# Autodesk Inventor assembly: Custom_Delta_Assembly
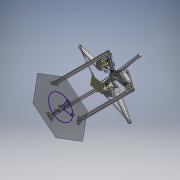
[picture p0: Inventor's stored thumbnail of the model, 180x180]
Saved by Autodesk Inventor 2019.4 (Build 234330000, 330)
## iProperties
Created: 2019-07-06
Part Number: Custom_Delta_Assembly
Document SubType Name: Assembly
Designer: Jorian Brusind
Author: Jorian Brusind
## Documents named in this file (16)
- C:\Users\Jorian Bruslind\Documents\GitHub\ECE44x_Senior_Design\Design files\Delta Robot Arm\Inventor Files\Custom_Delta\Custom_Delta_Assembly.iam
- C:\Users\Jorian Bruslind\Documents\GitHub\ECE44x_Senior_Design\Design files\Delta Robot Arm\Inventor Files\Custom_Delta\Stepper_Face.ipt
- C:\Users\Jorian Bruslind\Documents\GitHub\ECE44x_Senior_Design\Design files\Delta Robot Arm\Inventor Files\Custom_Delta\Delta_Arm.ipt
- C:\Users\Jorian Bruslind\Documents\GitHub\ECE44x_Senior_Design\Design files\Delta Robot Arm\Inventor Files\Custom_Delta\Delta_Top.ipt
- C:\Users\Jorian Bruslind\Documents\GitHub\ECE44x_Senior_Design\Design files\Delta Robot Arm\Inventor Files\McMaster Files\59935K140_METRIC BALL JOINT ROD END.ipt
- C:\Users\Jorian Bruslind\Documents\GitHub\ECE44x_Senior_Design\Design files\PetriFilm\PetriFilm.iam
- C:\Users\Jorian Bruslind\Documents\GitHub\ECE44x_Senior_Design\Design files\Delta Robot Arm\Inventor Files\McMaster Files\5537T501_ALUMINUM T-SLOTTED FRAMING EXTRUSION.ipt
- C:\Users\Jorian Bruslind\Documents\GitHub\ECE44x_Senior_Design\Design files\Delta Robot Arm\Inventor Files\McMaster Files\5537T518_T-SLOTTED FRAMING.ipt
- C:\Users\Jorian Bruslind\Documents\GitHub\ECE44x_Senior_Design\Design files\Delta Robot Arm\Inventor Files\McMaster Files\6In_ALUMINUM T-SLOTTED FRAMING EXTRUSION.ipt
- C:\Users\Jorian Bruslind\Documents\GitHub\ECE44x_Senior_Design\Design files\Delta Robot Arm\Inventor Files\McMaster Files\98861A050_LOW-STRENGTH STEEL THREADED ROD.ipt
- C:\Users\Jorian Bruslind\Documents\GitHub\ECE44x_Senior_Design\Design files\Delta Robot Arm\Inventor Files\Custom_Delta\Custom_Delta_End_Effector.ipt
- C:\Users\Jorian Bruslind\Documents\GitHub\ECE44x_Senior_Design\Design files\Delta Robot Arm\Inventor Files\Custom_Delta\80_20_Connector.ipt
- C:\Users\Jorian Bruslind\Documents\GitHub\ECE44x_Senior_Design\Design files\Delta Robot Arm\Inventor Files\Custom_Delta\NEMA17_Stepper_CL42H60.ipt
- C:\Users\Jorian Bruslind\Documents\GitHub\ECE44x_Senior_Design\Design files\Delta Robot Arm\Inventor Files\Stepper_Collar\products\12196\step\model.ipt
- C:\Users\Jorian Bruslind\Documents\GitHub\ECE44x_Senior_Design\Design files\Delta Robot Arm\Inventor Files\raspberry-pi-camera-module-v2-1.snapshot.3\RspCameraMia.iam
- C:\Users\Jorian Bruslind\Documents\GitHub\ECE44x_Senior_Design\Design files\Delta Robot Arm\Inventor Files\Custom_Delta\80_20_Connector_Bot.ipt
## Components (51 placed, 15 different names)
1. Stepper_Face:1 — Mate:126, Flush:20, Flush:23, Mate:210, Mate:211, Mate:212, Mate:216
2. Delta_Arm:1 — Mate:145, Mate:146, Mate:147, Mate:148, Mate:214, Mate:215, Mate:254
3. Stepper_Face:2 — Mate:125, Flush:18, Flush:24, Mate:222, Mate:227, Mate:230, Mate:231
4. Delta_Arm:2 — Mate:149, Mate:150, Mate:151, Mate:152, Mate:220, Mate:221, Mate:253
5. Stepper_Face:3 — Mate:127, Flush:21, Flush:22, Mate:217, Mate:218, Mate:226, Mate:228
6. Delta_Arm:3 — Mate:137, Mate:138, Mate:139, Mate:140, Mate:224, Mate:225, Mate:229
7. Delta_Top:1 — Mate:103, Mate:105, Mate:106, Mate:107, Mate:109, Mate:110, Mate:111, Mate:112, Mate:113, Mate:182, Mate:189, Mate:190, Mate:191, Mate:192, Mate:238, Mate:240, Mate:241, Mate:243, Mate:244, Mate:246
8. 59935K140_METRIC BALL JOINT ROD END:2 — Mate:145, Mate:146, Mate:159, Mate:160
9. 59935K140_METRIC BALL JOINT ROD END:3 — Mate:151, Mate:152, Mate:153, Mate:154
10. 59935K140_METRIC BALL JOINT ROD END:5 — Mate:137, Mate:138, Mate:143, Mate:144
11. 59935K140_METRIC BALL JOINT ROD END:6 — Mate:139, Mate:140, Mate:141, Mate:142
12. 59935K140_METRIC BALL JOINT ROD END:7 — Mate:147, Mate:148, Mate:157, Mate:158
13. 59935K140_METRIC BALL JOINT ROD END:8 — Mate:149, Mate:150, Mate:155, Mate:156
14. PetriFilm:1 [sub-assembly] — Mate:181, Mate:183
15. 5537T518_T-SLOTTED FRAMING:1 — Mate:106, Mate:107, Mate:119
16. 5537T518_T-SLOTTED FRAMING:2 — Mate:103, Mate:105, Mate:118
17. 5537T518_T-SLOTTED FRAMING:3 — Mate:109, Mate:110, Mate:117
18. 6In_ALUMINUM T-SLOTTED FRAMING EXTRUSION:1 — Flush:5, Mate:121, Flush:6, Mate:126, Flush:20, Flush:23, Mate:188, Mate:235, Mate:247
19. 6In_ALUMINUM T-SLOTTED FRAMING EXTRUSION:2 — Flush:9, Flush:10, Mate:123, Mate:125, Flush:18, Flush:24, Mate:237
20. 6In_ALUMINUM T-SLOTTED FRAMING EXTRUSION:3 — Flush:7, Flush:8, Mate:122, Mate:127, Flush:21, Flush:22, Mate:233
21. 5537T501_ALUMINUM T-SLOTTED FRAMING EXTRUSION:1 — Mate:112, Mate:118, Flush:5, Mate:121, Flush:6, Mate:192, Mate:234, Flush:26, Mate:245
22. 5537T501_ALUMINUM T-SLOTTED FRAMING EXTRUSION:2 — Mate:111, Mate:119, Flush:7, Flush:8, Mate:122, Mate:190, Mate:232, Flush:25, Mate:239
23. 5537T501_ALUMINUM T-SLOTTED FRAMING EXTRUSION:3 — Mate:113, Mate:117, Flush:9, Flush:10, Mate:123, Mate:191, Mate:236, Flush:27, Mate:242
24. 98861A050_LOW-STRENGTH STEEL THREADED ROD:1 — Mate:143, Mate:144, Mate:163, Mate:164
25. 98861A050_LOW-STRENGTH STEEL THREADED ROD:2 — Mate:153, Mate:154, Mate:168, Mate:170
26. 98861A050_LOW-STRENGTH STEEL THREADED ROD:3 — Mate:155, Mate:156, Mate:167, Mate:169
27. 98861A050_LOW-STRENGTH STEEL THREADED ROD:4 — Mate:141, Mate:142, Mate:161, Mate:162
28. 98861A050_LOW-STRENGTH STEEL THREADED ROD:5 — Mate:157, Mate:158, Mate:165, Mate:172
29. 98861A050_LOW-STRENGTH STEEL THREADED ROD:6 — Mate:159, Mate:160, Mate:166, Mate:171
30. 59935K140_METRIC BALL JOINT ROD END:9 — Mate:165, Mate:172, Mate:174, Mate:178
31. 59935K140_METRIC BALL JOINT ROD END:10 — Mate:163, Mate:164, Mate:176
32. 59935K140_METRIC BALL JOINT ROD END:11 — Mate:166, Mate:171, Mate:174
33. 59935K140_METRIC BALL JOINT ROD END:12 — Mate:161, Mate:162, Mate:176, Mate:180
34. 59935K140_METRIC BALL JOINT ROD END:13 — Mate:168, Mate:170, Mate:175
35. 59935K140_METRIC BALL JOINT ROD END:14 — Mate:167, Mate:169, Mate:175, Mate:179
36. Custom_Delta_End_Effector:1 — Mate:178, Mate:179, Mate:180, Mate:181, Mate:182, Mate:183
37. 80_20_Connector:1 — Mate:188, Mate:189, Mate:248, Mate:249
38. NEMA17_Stepper_CL42H60:1 — Mate:219, Mate:227, Mate:230, Mate:231
39. NEMA17_Stepper_CL42H60:2 — Mate:210, Mate:211, Mate:212, Mate:213
40. NEMA17_Stepper_CL42H60:3 — Mate:217, Mate:218, Mate:223, Mate:228
41. model:4 — Mate:223, Mate:224, Mate:225, Mate:226, Mate:229
42. model:5 — Mate:213, Mate:214, Mate:215, Mate:216, Mate:254
43. model:6 — Mate:219, Mate:220, Mate:221, Mate:222, Mate:253
44. 5537T518_T-SLOTTED FRAMING:4 — Mate:236, Mate:237, Flush:27
45. 5537T518_T-SLOTTED FRAMING:5 — Mate:232, Mate:233, Flush:25
46. 5537T518_T-SLOTTED FRAMING:6 — Mate:234, Mate:235, Flush:26
47. 5537T518_T-SLOTTED FRAMING:7 — Mate:238, Mate:239, Mate:240
48. 5537T518_T-SLOTTED FRAMING:8 — Mate:241, Mate:242, Mate:243
49. 5537T518_T-SLOTTED FRAMING:9 — Mate:244, Mate:245, Mate:246
50. RspCameraMia:1 [sub-assembly] — Mate:250, Mate:251, Mate:252
51. 80_20_Connector_Bot:1 — Mate:247, Mate:248, Mate:249, Mate:250, Mate:251, Mate:252
## Relationships (128: Mate 113, Flush 15)
- Mate:103: Delta_Top:1 ↔ 5537T518_T-SLOTTED FRAMING:2
- Mate:105: Delta_Top:1 ↔ 5537T518_T-SLOTTED FRAMING:2
- Mate:106: Delta_Top:1 ↔ 5537T518_T-SLOTTED FRAMING:1
- Mate:107: Delta_Top:1 ↔ 5537T518_T-SLOTTED FRAMING:1
- Mate:109: Delta_Top:1 ↔ 5537T518_T-SLOTTED FRAMING:3
- Mate:110: Delta_Top:1 ↔ 5537T518_T-SLOTTED FRAMING:3
- Mate:111: Delta_Top:1 ↔ 5537T501_ALUMINUM T-SLOTTED FRAMING EXTRUSION:2
- Mate:112: Delta_Top:1 ↔ 5537T501_ALUMINUM T-SLOTTED FRAMING EXTRUSION:1
- Mate:113: Delta_Top:1 ↔ 5537T501_ALUMINUM T-SLOTTED FRAMING EXTRUSION:3
- Mate:117: 5537T518_T-SLOTTED FRAMING:3 ↔ 5537T501_ALUMINUM T-SLOTTED FRAMING EXTRUSION:3
- Mate:118: 5537T518_T-SLOTTED FRAMING:2 ↔ 5537T501_ALUMINUM T-SLOTTED FRAMING EXTRUSION:1
- Mate:119: 5537T518_T-SLOTTED FRAMING:1 ↔ 5537T501_ALUMINUM T-SLOTTED FRAMING EXTRUSION:2
- Flush:5: 6In_ALUMINUM T-SLOTTED FRAMING EXTRUSION:1 ↔ 5537T501_ALUMINUM T-SLOTTED FRAMING EXTRUSION:1
- Mate:121: 6In_ALUMINUM T-SLOTTED FRAMING EXTRUSION:1 ↔ 5537T501_ALUMINUM T-SLOTTED FRAMING EXTRUSION:1
- Flush:6: 6In_ALUMINUM T-SLOTTED FRAMING EXTRUSION:1 ↔ 5537T501_ALUMINUM T-SLOTTED FRAMING EXTRUSION:1
- Flush:7: 6In_ALUMINUM T-SLOTTED FRAMING EXTRUSION:3 ↔ 5537T501_ALUMINUM T-SLOTTED FRAMING EXTRUSION:2
- Flush:8: 6In_ALUMINUM T-SLOTTED FRAMING EXTRUSION:3 ↔ 5537T501_ALUMINUM T-SLOTTED FRAMING EXTRUSION:2
- Mate:122: 6In_ALUMINUM T-SLOTTED FRAMING EXTRUSION:3 ↔ 5537T501_ALUMINUM T-SLOTTED FRAMING EXTRUSION:2
- Flush:9: 6In_ALUMINUM T-SLOTTED FRAMING EXTRUSION:2 ↔ 5537T501_ALUMINUM T-SLOTTED FRAMING EXTRUSION:3
- Flush:10: 6In_ALUMINUM T-SLOTTED FRAMING EXTRUSION:2 ↔ 5537T501_ALUMINUM T-SLOTTED FRAMING EXTRUSION:3
- Mate:123: 6In_ALUMINUM T-SLOTTED FRAMING EXTRUSION:2 ↔ 5537T501_ALUMINUM T-SLOTTED FRAMING EXTRUSION:3
- Mate:125: Stepper_Face:2 ↔ 6In_ALUMINUM T-SLOTTED FRAMING EXTRUSION:2
- Mate:126: Stepper_Face:1 ↔ 6In_ALUMINUM T-SLOTTED FRAMING EXTRUSION:1
- Mate:127: Stepper_Face:3 ↔ 6In_ALUMINUM T-SLOTTED FRAMING EXTRUSION:3
- Mate:137: Delta_Arm:3 ↔ 59935K140_METRIC BALL JOINT ROD END:5
- Mate:138: Delta_Arm:3 ↔ 59935K140_METRIC BALL JOINT ROD END:5
- Mate:139: Delta_Arm:3 ↔ 59935K140_METRIC BALL JOINT ROD END:6
- Mate:140: Delta_Arm:3 ↔ 59935K140_METRIC BALL JOINT ROD END:6
- Mate:141: 59935K140_METRIC BALL JOINT ROD END:6 ↔ 98861A050_LOW-STRENGTH STEEL THREADED ROD:4
- Mate:142: 59935K140_METRIC BALL JOINT ROD END:6 ↔ 98861A050_LOW-STRENGTH STEEL THREADED ROD:4
- Mate:143: 59935K140_METRIC BALL JOINT ROD END:5 ↔ 98861A050_LOW-STRENGTH STEEL THREADED ROD:1
- Mate:144: 59935K140_METRIC BALL JOINT ROD END:5 ↔ 98861A050_LOW-STRENGTH STEEL THREADED ROD:1
- Mate:145: Delta_Arm:1 ↔ 59935K140_METRIC BALL JOINT ROD END:2
- Mate:146: Delta_Arm:1 ↔ 59935K140_METRIC BALL JOINT ROD END:2
- Mate:147: Delta_Arm:1 ↔ 59935K140_METRIC BALL JOINT ROD END:7
- Mate:148: Delta_Arm:1 ↔ 59935K140_METRIC BALL JOINT ROD END:7
- Mate:149: Delta_Arm:2 ↔ 59935K140_METRIC BALL JOINT ROD END:8
- Mate:150: Delta_Arm:2 ↔ 59935K140_METRIC BALL JOINT ROD END:8
- Mate:151: Delta_Arm:2 ↔ 59935K140_METRIC BALL JOINT ROD END:3
- Mate:152: Delta_Arm:2 ↔ 59935K140_METRIC BALL JOINT ROD END:3
- Mate:153: 59935K140_METRIC BALL JOINT ROD END:3 ↔ 98861A050_LOW-STRENGTH STEEL THREADED ROD:2
- Mate:154: 59935K140_METRIC BALL JOINT ROD END:3 ↔ 98861A050_LOW-STRENGTH STEEL THREADED ROD:2
- Mate:155: 59935K140_METRIC BALL JOINT ROD END:8 ↔ 98861A050_LOW-STRENGTH STEEL THREADED ROD:3
- Mate:156: 59935K140_METRIC BALL JOINT ROD END:8 ↔ 98861A050_LOW-STRENGTH STEEL THREADED ROD:3
- Mate:157: 59935K140_METRIC BALL JOINT ROD END:7 ↔ 98861A050_LOW-STRENGTH STEEL THREADED ROD:5
- Mate:158: 59935K140_METRIC BALL JOINT ROD END:7 ↔ 98861A050_LOW-STRENGTH STEEL THREADED ROD:5
- Mate:159: 59935K140_METRIC BALL JOINT ROD END:2 ↔ 98861A050_LOW-STRENGTH STEEL THREADED ROD:6
- Mate:160: 59935K140_METRIC BALL JOINT ROD END:2 ↔ 98861A050_LOW-STRENGTH STEEL THREADED ROD:6
- Mate:161: 98861A050_LOW-STRENGTH STEEL THREADED ROD:4 ↔ 59935K140_METRIC BALL JOINT ROD END:12
- Mate:162: 98861A050_LOW-STRENGTH STEEL THREADED ROD:4 ↔ 59935K140_METRIC BALL JOINT ROD END:12
- Mate:163: 98861A050_LOW-STRENGTH STEEL THREADED ROD:1 ↔ 59935K140_METRIC BALL JOINT ROD END:10
- Mate:164: 98861A050_LOW-STRENGTH STEEL THREADED ROD:1 ↔ 59935K140_METRIC BALL JOINT ROD END:10
- Mate:165: 98861A050_LOW-STRENGTH STEEL THREADED ROD:5 ↔ 59935K140_METRIC BALL JOINT ROD END:9
- Mate:166: 98861A050_LOW-STRENGTH STEEL THREADED ROD:6 ↔ 59935K140_METRIC BALL JOINT ROD END:11
- Mate:167: 98861A050_LOW-STRENGTH STEEL THREADED ROD:3 ↔ 59935K140_METRIC BALL JOINT ROD END:14
- Mate:168: 98861A050_LOW-STRENGTH STEEL THREADED ROD:2 ↔ 59935K140_METRIC BALL JOINT ROD END:13
- Mate:169: 98861A050_LOW-STRENGTH STEEL THREADED ROD:3 ↔ 59935K140_METRIC BALL JOINT ROD END:14
- Mate:170: 98861A050_LOW-STRENGTH STEEL THREADED ROD:2 ↔ 59935K140_METRIC BALL JOINT ROD END:13
- Mate:171: 98861A050_LOW-STRENGTH STEEL THREADED ROD:6 ↔ 59935K140_METRIC BALL JOINT ROD END:11
- Mate:172: 98861A050_LOW-STRENGTH STEEL THREADED ROD:5 ↔ 59935K140_METRIC BALL JOINT ROD END:9
- Mate:174: 59935K140_METRIC BALL JOINT ROD END:9 ↔ 59935K140_METRIC BALL JOINT ROD END:11
- Mate:175: 59935K140_METRIC BALL JOINT ROD END:13 ↔ 59935K140_METRIC BALL JOINT ROD END:14
- Mate:176: 59935K140_METRIC BALL JOINT ROD END:10 ↔ 59935K140_METRIC BALL JOINT ROD END:12
- Flush:18: Stepper_Face:2 ↔ 6In_ALUMINUM T-SLOTTED FRAMING EXTRUSION:2
- Flush:20: Stepper_Face:1 ↔ 6In_ALUMINUM T-SLOTTED FRAMING EXTRUSION:1
- Flush:21: Stepper_Face:3 ↔ 6In_ALUMINUM T-SLOTTED FRAMING EXTRUSION:3
- Flush:22 (112.406 mm): Stepper_Face:3 ↔ 6In_ALUMINUM T-SLOTTED FRAMING EXTRUSION:3
- Flush:23 (112.206 mm): Stepper_Face:1 ↔ 6In_ALUMINUM T-SLOTTED FRAMING EXTRUSION:1
- Flush:24 (112.406 mm): Stepper_Face:2 ↔ 6In_ALUMINUM T-SLOTTED FRAMING EXTRUSION:2
- Mate:178: 59935K140_METRIC BALL JOINT ROD END:9 ↔ Custom_Delta_End_Effector:1
- Mate:179: 59935K140_METRIC BALL JOINT ROD END:14 ↔ Custom_Delta_End_Effector:1
- Mate:180: 59935K140_METRIC BALL JOINT ROD END:12 ↔ Custom_Delta_End_Effector:1
- Mate:181: PetriFilm:1 ↔ Custom_Delta_End_Effector:1
- Mate:182: Delta_Top:1 ↔ Custom_Delta_End_Effector:1
- Mate:183 (-25 mm): PetriFilm:1 ↔ Custom_Delta_End_Effector:1
- Mate:188: 6In_ALUMINUM T-SLOTTED FRAMING EXTRUSION:1 ↔ 80_20_Connector:1
- Mate:189: Delta_Top:1 ↔ 80_20_Connector:1
- Mate:190: Delta_Top:1 ↔ 5537T501_ALUMINUM T-SLOTTED FRAMING EXTRUSION:2
- Mate:191: Delta_Top:1 ↔ 5537T501_ALUMINUM T-SLOTTED FRAMING EXTRUSION:3
- Mate:192: Delta_Top:1 ↔ 5537T501_ALUMINUM T-SLOTTED FRAMING EXTRUSION:1
- Mate:210: Stepper_Face:1 ↔ NEMA17_Stepper_CL42H60:2
- Mate:211: Stepper_Face:1 ↔ NEMA17_Stepper_CL42H60:2
- Mate:212: Stepper_Face:1 ↔ NEMA17_Stepper_CL42H60:2
- Mate:213: NEMA17_Stepper_CL42H60:2 ↔ model:5
- Mate:214: Delta_Arm:1 ↔ model:5
- Mate:215: Delta_Arm:1 ↔ model:5
- Mate:216: Stepper_Face:1 ↔ model:5
- Mate:217: Stepper_Face:3 ↔ NEMA17_Stepper_CL42H60:3
- Mate:218: Stepper_Face:3 ↔ NEMA17_Stepper_CL42H60:3
- Mate:219: NEMA17_Stepper_CL42H60:1 ↔ model:6
- Mate:220: Delta_Arm:2 ↔ model:6
- Mate:221: Delta_Arm:2 ↔ model:6
- Mate:222: Stepper_Face:2 ↔ model:6
- Mate:223: NEMA17_Stepper_CL42H60:3 ↔ model:4
- Mate:224: Delta_Arm:3 ↔ model:4
- Mate:225: Delta_Arm:3 ↔ model:4
- Mate:226: Stepper_Face:3 ↔ model:4
- Mate:227: Stepper_Face:2 ↔ NEMA17_Stepper_CL42H60:1
- Mate:228: Stepper_Face:3 ↔ NEMA17_Stepper_CL42H60:3
- Mate:229: Delta_Arm:3 ↔ model:4
- Mate:230: Stepper_Face:2 ↔ NEMA17_Stepper_CL42H60:1
- Mate:231: Stepper_Face:2 ↔ NEMA17_Stepper_CL42H60:1
- Mate:232: 5537T501_ALUMINUM T-SLOTTED FRAMING EXTRUSION:2 ↔ 5537T518_T-SLOTTED FRAMING:5
- Mate:233: 6In_ALUMINUM T-SLOTTED FRAMING EXTRUSION:3 ↔ 5537T518_T-SLOTTED FRAMING:5
- Flush:25: 5537T501_ALUMINUM T-SLOTTED FRAMING EXTRUSION:2 ↔ 5537T518_T-SLOTTED FRAMING:5
- Mate:234: 5537T501_ALUMINUM T-SLOTTED FRAMING EXTRUSION:1 ↔ 5537T518_T-SLOTTED FRAMING:6
- Mate:235: 6In_ALUMINUM T-SLOTTED FRAMING EXTRUSION:1 ↔ 5537T518_T-SLOTTED FRAMING:6
- Flush:26: 5537T501_ALUMINUM T-SLOTTED FRAMING EXTRUSION:1 ↔ 5537T518_T-SLOTTED FRAMING:6
- Mate:236: 5537T501_ALUMINUM T-SLOTTED FRAMING EXTRUSION:3 ↔ 5537T518_T-SLOTTED FRAMING:4
- Mate:237: 6In_ALUMINUM T-SLOTTED FRAMING EXTRUSION:2 ↔ 5537T518_T-SLOTTED FRAMING:4
- Flush:27: 5537T501_ALUMINUM T-SLOTTED FRAMING EXTRUSION:3 ↔ 5537T518_T-SLOTTED FRAMING:4
- Mate:238: Delta_Top:1 ↔ 5537T518_T-SLOTTED FRAMING:7
- Mate:239: 5537T501_ALUMINUM T-SLOTTED FRAMING EXTRUSION:2 ↔ 5537T518_T-SLOTTED FRAMING:7
- Mate:240: Delta_Top:1 ↔ 5537T518_T-SLOTTED FRAMING:7
- Mate:241: Delta_Top:1 ↔ 5537T518_T-SLOTTED FRAMING:8
- Mate:242: 5537T501_ALUMINUM T-SLOTTED FRAMING EXTRUSION:3 ↔ 5537T518_T-SLOTTED FRAMING:8
- Mate:243: Delta_Top:1 ↔ 5537T518_T-SLOTTED FRAMING:8
- Mate:244: Delta_Top:1 ↔ 5537T518_T-SLOTTED FRAMING:9
- Mate:245: 5537T501_ALUMINUM T-SLOTTED FRAMING EXTRUSION:1 ↔ 5537T518_T-SLOTTED FRAMING:9
- Mate:246: Delta_Top:1 ↔ 5537T518_T-SLOTTED FRAMING:9
- Mate:247: 6In_ALUMINUM T-SLOTTED FRAMING EXTRUSION:1 ↔ 80_20_Connector_Bot:1
- Mate:248: 80_20_Connector:1 ↔ 80_20_Connector_Bot:1
- Mate:249: 80_20_Connector:1 ↔ 80_20_Connector_Bot:1
- Mate:250: RspCameraMia:1 ↔ 80_20_Connector_Bot:1
- Mate:251: RspCameraMia:1 ↔ 80_20_Connector_Bot:1
- Mate:252: RspCameraMia:1 ↔ 80_20_Connector_Bot:1
- Mate:253: Delta_Arm:2 ↔ model:6
- Mate:254: Delta_Arm:1 ↔ model:5
